# Autodesk Inventor assembly: licht_200
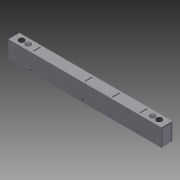
[picture p0: Inventor's stored thumbnail of the model, 180x180]
Saved by Autodesk Inventor 2015 (Build 190159000, 159)
## iProperties
Created: 2018-02-17
Part Number: licht_200
Document SubType Name: Assembly
Designer: wepet
Author: wepet
## Documents named in this file (13)
- C:\workspace\robosax\licht\Einzelteil_150\licht_150.iam
- C:\workspace\robosax\licht\Einzelteil_150\licht_150_back.ipt
- C:\workspace\robosax\licht\Einzelteil_150\licht_150_front.ipt
- C:\workspace\robosax\licht\Einzelteil_150\licht_150_top.ipt
- C:\workspace\robosax\licht\Einzelteil_150\licht_150_side_middle.ipt
- C:\workspace\robosax\licht\Zusatzelemente\licht_led_blau.ipt
- C:\workspace\robosax\licht\Zusatzelemente\licht_taster.ipt
- C:\workspace\robosax\licht\Zusatzelemente\anschluss_strom.ipt
- C:\workspace\robosax\licht\Zusatzelemente\anschluss_daten.iam
- C:\workspace\robosax\licht\Einzelteil_150\licht_150_side_right.ipt
- C:\workspace\robosax\licht\Einzelteil_150\licht_150_side_left.ipt
- C:\workspace\robosax\licht\Einzelteil_150\licht_150_support_right.ipt
- C:\workspace\robosax\licht\Einzelteil_150\licht_150_support_left.ipt
## Components (20 placed, 12 different names)
1. licht_150_back:1 — Fluchtend:3, Fluchtend:4, Fluchtend:5, Passend:9, Fluchtend:13
2. licht_150_front:1 — Passend:1, Passend:2, Passend:3, Passend:4, Fluchtend:1, Fluchtend:2, Fluchtend:3, Fluchtend:4, Passend:10, Einfügen:1, Einfügen:2, Einfügen:3, Einfügen:4, Einfügen:5, Einfügen:6, Einfügen:7, Einfügen:8, Passend:36, Passend:37, Fluchtend:12, Passend:39, Passend:42, Passend:45
3. licht_150_top:1 — Passend:4, Fluchtend:1, Fluchtend:2, Fluchtend:5, Passend:8, Drehbar:1, Passend:26, Passend:27, Passend:28, Passend:29, Passend:30, Passend:31, Passend:32, Passend:33, Passend:34, Passend:38, Passend:40, Passend:41, Passend:44
4. licht_150_side_middle:1 — Passend:8, Passend:9, Passend:10, Passend:36
5. licht_led_blau:1 — Einfügen:4
6. licht_led_blau:2 — Einfügen:3
7. licht_led_blau:3 — Einfügen:1
8. licht_led_blau:4 — Einfügen:2
9. licht_taster:1 — Einfügen:5
10. licht_taster:2 — Einfügen:6
11. licht_taster:3 — Einfügen:7
12. licht_taster:4 — Einfügen:8
13. anschluss_strom:1 — Drehbar:1, Passend:26
14. anschluss_strom:2 — Passend:30, Passend:31
15. anschluss_daten:1 [sub-assembly] — Passend:27, Passend:28, Passend:29
16. anschluss_daten:2 [sub-assembly] — Passend:32, Passend:33, Passend:34
17. licht_150_side_right:1 — Passend:37, Fluchtend:12, Passend:38, Passend:43
18. licht_150_side_left:1 — Passend:39, Passend:40, Fluchtend:13, Passend:46
19. licht_150_support_right:1 — Passend:41, Passend:42, Passend:43
20. licht_150_support_left:1 — Passend:44, Passend:45, Passend:46
## Relationships (43: Mate 27, Insert 8, Flush 7, RevoluteJoint 1)
- Passend:1 [Mate]: licht_150_front:1
- Passend:2 [Mate]: licht_150_front:1
- Passend:3 [Mate]: licht_150_front:1
- Passend:4 [Mate]: licht_150_front:1 ↔ licht_150_top:1
- Fluchtend:1 [Flush]: licht_150_front:1 ↔ licht_150_top:1
- Fluchtend:2 [Flush]: licht_150_front:1 ↔ licht_150_top:1
- Fluchtend:3 [Flush]: licht_150_back:1 ↔ licht_150_front:1
- Fluchtend:4 [Flush]: licht_150_back:1 ↔ licht_150_front:1
- Fluchtend:5 [Flush]: licht_150_back:1 ↔ licht_150_top:1
- Passend:8 [Mate]: licht_150_top:1 ↔ licht_150_side_middle:1
- Passend:9 [Mate]: licht_150_back:1 ↔ licht_150_side_middle:1
- Passend:10 [Mate]: licht_150_front:1 ↔ licht_150_side_middle:1
- Einfügen:1 [Insert] (-5 mm): licht_150_front:1 ↔ licht_led_blau:3
- Einfügen:2 [Insert] (-5 mm): licht_150_front:1 ↔ licht_led_blau:4
- Einfügen:3 [Insert]: licht_150_front:1 ↔ licht_led_blau:2
- Einfügen:4 [Insert]: licht_150_front:1 ↔ licht_led_blau:1
- Einfügen:5 [Insert] (5 mm): licht_150_front:1 ↔ licht_taster:1
- Einfügen:6 [Insert] (5 mm): licht_150_front:1 ↔ licht_taster:2
- Einfügen:7 [Insert] (5 mm): licht_150_front:1 ↔ licht_taster:3
- Einfügen:8 [Insert] (5 mm): licht_150_front:1 ↔ licht_taster:4
- Drehbar:1 [RevoluteJoint] (-7 mm): licht_150_top:1 ↔ anschluss_strom:1
- Passend:26 [Mate]: licht_150_top:1 ↔ anschluss_strom:1
- Passend:27 [Mate]: licht_150_top:1 ↔ anschluss_daten:1
- Passend:28 [Mate]: licht_150_top:1 ↔ anschluss_daten:1
- Passend:29 [Mate]: licht_150_top:1 ↔ anschluss_daten:1
- Passend:30 [Mate]: licht_150_top:1 ↔ anschluss_strom:2
- Passend:31 [Mate]: licht_150_top:1 ↔ anschluss_strom:2
- Passend:32 [Mate]: licht_150_top:1 ↔ anschluss_daten:2
- Passend:33 [Mate]: licht_150_top:1 ↔ anschluss_daten:2
- Passend:34 [Mate]: licht_150_top:1 ↔ anschluss_daten:2
- Passend:36 [Mate]: licht_150_front:1 ↔ licht_150_side_middle:1
- Passend:37 [Mate]: licht_150_front:1 ↔ licht_150_side_right:1
- Fluchtend:12 [Flush]: licht_150_front:1 ↔ licht_150_side_right:1
- Passend:38 [Mate]: licht_150_top:1 ↔ licht_150_side_right:1
- Passend:39 [Mate]: licht_150_front:1 ↔ licht_150_side_left:1
- Passend:40 [Mate]: licht_150_top:1 ↔ licht_150_side_left:1
- Fluchtend:13 [Flush]: licht_150_back:1 ↔ licht_150_side_left:1
- Passend:41 [Mate]: licht_150_top:1 ↔ licht_150_support_right:1
- Passend:42 [Mate]: licht_150_front:1 ↔ licht_150_support_right:1
- Passend:43 [Mate]: licht_150_side_right:1 ↔ licht_150_support_right:1
- Passend:44 [Mate]: licht_150_top:1 ↔ licht_150_support_left:1
- Passend:45 [Mate]: licht_150_front:1 ↔ licht_150_support_left:1
- Passend:46 [Mate]: licht_150_side_left:1 ↔ licht_150_support_left:1
